# Autodesk Inventor assembly: A100EnsembleCenteringDevice
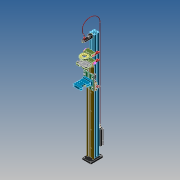
[picture p0: Inventor's stored thumbnail of the model, 180x180]
Saved by Autodesk Inventor 2020 (Build 240168000, 168)
## iProperties
Created: 2016-06-02
Part Number: A100EnsembleCenteringDevice
Document SubType Name: Assembly
Designer: serge.amoos
Author: serge.amoos
## Documents named in this file (15)
- R:\Diploma\TD2021\SYND\brice.dubuis\Hardware\pièces mécaniques\FocalMeasure\A100EnsembleFocalMeasure.iam
- R:\Diploma\TD2021\SYND\brice.dubuis\Hardware\pièces mécaniques\FocalMeasure\P101PlaqueDeBase.ipt
- R:\Diploma\TD2021\SYND\brice.dubuis\Hardware\pièces mécaniques\FocalMeasure\P100Colonne.ipt
- R:\Diploma\TD2021\SYND\brice.dubuis\Hardware\pièces mécaniques\FocalMeasure\F101IgusRailWS10x40x600.ipt
- R:\Diploma\TD2021\SYND\brice.dubuis\Hardware\pièces mécaniques\FocalMeasure\F102IgusPatinWW10x40x10HKA.ipt
- R:\Diploma\TD2021\SYND\brice.dubuis\Hardware\pièces mécaniques\FocalMeasure\A101EnsembleChariot.iam
- R:\Diploma\TD2021\SYND\brice.dubuis\Hardware\pièces mécaniques\FocalMeasure\P108EntretoiseCamera.ipt
- R:\Diploma\TD2021\SYND\brice.dubuis\Hardware\pièces mécaniques\FocalMeasure\A102EnsembleCamera.iam
- R:\Diploma\TD2021\SYND\brice.dubuis\Hardware\pièces mécaniques\FocalMeasure\F104ViTcyl6pcM3x16.ipt
- R:\Diploma\TD2021\SYND\brice.dubuis\Hardware\pièces mécaniques\FocalMeasure\A103EnsembleChariotCarre.iam
- R:\Diploma\TD2021\SYND\brice.dubuis\Hardware\pièces mécaniques\FocalMeasure\P116SupportFibre.ipt
- R:\Diploma\TD2021\SYND\brice.dubuis\Hardware\pièces mécaniques\FocalMeasure\F108VisTcyl6pcM6x30.ipt
- R:\Diploma\TD2021\SYND\brice.dubuis\Hardware\pièces mécaniques\FocalMeasure\F109VisTcyl6pcM8x20.ipt
- R:\Diploma\TD2021\SYND\brice.dubuis\Hardware\pièces mécaniques\FocalMeasure\F118Laser.ipt
- R:\Diploma\TD2021\SYND\brice.dubuis\Hardware\pièces mécaniques\FocalMeasure\A104EnsembleBoitierLaser.iam
## Components (15 placed, 14 different names)
1. P101PlaqueDeBase:1 — Mate:1, Mate:2, Flush:4, Insert:4
2. P100Colonne:1 — Mate:1, Mate:2, Flush:4, Mate:3, Flush:6, Flush:7, Mate:16, Mate:6, Mate:13, Mate:14, Mate:15, Mate:17, Mate:18, Flush:8, Mate:21
3. F101IgusRailWS10x40x600:1 — Mate:3, Mate:4, Mate:5, Flush:6, Flush:7
4. F102IgusPatinWW10x40x10HKA:1 — Mate:4, Mate:5, Mate:11, Mate:12, Mate:19
5. A101EnsembleChariot:1 [sub-assembly] — Mate:16, Mate:6
6. P108EntretoiseCamera:1 — Mate:7, Mate:8, Mate:9, Mate:11, Mate:12, Insert:1, Insert:2, Mate:19
7. A102EnsembleCamera:1 [sub-assembly] — Mate:7, Mate:8, Mate:9
8. F104ViTcyl6pcM3x16:1 — Insert:2
9. F104ViTcyl6pcM3x16:2 — Insert:1
10. A103EnsembleChariotCarre:1 [sub-assembly] — Mate:13, Mate:14
11. P116SupportFibre:1 — Mate:15, Insert:3, Mate:20, Flush:8, Mate:21
12. F108VisTcyl6pcM6x30:1 — Insert:3
13. F109VisTcyl6pcM8x20:1 — Insert:4
14. A104EnsembleBoitierLaser:1 [sub-assembly] — Mate:17, Mate:18
15. F118Laser:1 — Mate:20
## Relationships (28: Mate 20, Flush 4, Insert 4)
- Mate:1: P101PlaqueDeBase:1 ↔ P100Colonne:1
- Mate:2: P101PlaqueDeBase:1 ↔ P100Colonne:1
- Flush:4: P101PlaqueDeBase:1 ↔ P100Colonne:1
- Mate:3: P100Colonne:1 ↔ F101IgusRailWS10x40x600:1
- Mate:4: F101IgusRailWS10x40x600:1 ↔ F102IgusPatinWW10x40x10HKA:1
- Mate:5: F101IgusRailWS10x40x600:1 ↔ F102IgusPatinWW10x40x10HKA:1
- Flush:6: P100Colonne:1 ↔ F101IgusRailWS10x40x600:1
- Flush:7: P100Colonne:1 ↔ F101IgusRailWS10x40x600:1
- Mate:16: P100Colonne:1 ↔ A101EnsembleChariot:1
- Mate:6: P100Colonne:1 ↔ A101EnsembleChariot:1
- Mate:7: P108EntretoiseCamera:1 ↔ A102EnsembleCamera:1
- Mate:8: P108EntretoiseCamera:1 ↔ A102EnsembleCamera:1
- Mate:9: P108EntretoiseCamera:1 ↔ A102EnsembleCamera:1
- Mate:11: F102IgusPatinWW10x40x10HKA:1 ↔ P108EntretoiseCamera:1
- Mate:12: F102IgusPatinWW10x40x10HKA:1 ↔ P108EntretoiseCamera:1
- Insert:1: P108EntretoiseCamera:1 ↔ F104ViTcyl6pcM3x16:2
- Insert:2: P108EntretoiseCamera:1 ↔ F104ViTcyl6pcM3x16:1
- Mate:13: P100Colonne:1 ↔ A103EnsembleChariotCarre:1
- Mate:14: P100Colonne:1 ↔ A103EnsembleChariotCarre:1
- Mate:15: P100Colonne:1 ↔ P116SupportFibre:1
- Insert:3: P116SupportFibre:1 ↔ F108VisTcyl6pcM6x30:1
- Insert:4: P101PlaqueDeBase:1 ↔ F109VisTcyl6pcM8x20:1
- Mate:17: P100Colonne:1 ↔ A104EnsembleBoitierLaser:1
- Mate:18: P100Colonne:1 ↔ A104EnsembleBoitierLaser:1
- Mate:19: F102IgusPatinWW10x40x10HKA:1 ↔ P108EntretoiseCamera:1
- Mate:20: P116SupportFibre:1 ↔ F118Laser:1
- Flush:8: P100Colonne:1 ↔ P116SupportFibre:1
- Mate:21: P100Colonne:1 ↔ P116SupportFibre:1
